# Autodesk Inventor assembly: Ensemble support
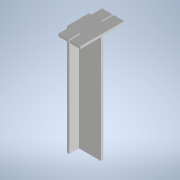
[picture p0: Inventor's stored thumbnail of the model, 180x180]
Saved by Autodesk Inventor 2020 (Build 240168000, 168)
## iProperties
Created: 2019-11-07
Part Number: Ensemble support
Document SubType Name: Assembly
Designer: change_le_nom
Author: change_le_nom
## Documents named in this file (4)
- D:\EIRBOT\Coupe de France 2020\Table de jeu\Support de balise centrale\Ensemble support.iam
- D:\EIRBOT\Coupe de France 2020\Table de jeu\Support de balise centrale\Pièce1.ipt
- D:\EIRBOT\Coupe de France 2020\Table de jeu\Support de balise centrale\Pièce2.ipt
- D:\EIRBOT\Coupe de France 2020\Table de jeu\Support de balise centrale\Pièce3.ipt
## Components (3 placed, 3 different names)
1. Pièce1:1 — Placage:1, Placage:2, Placage:3, Affleurement:1, Affleurement:2, Placage:5, Placage:6
2. Pièce2:1 — Placage:3, Affleurement:1, Affleurement:2, Placage:4
3. Pièce3:1 — Placage:4, Placage:5, Placage:6
## Relationships (8: Mate 6, Flush 2)
- Placage:1 [Mate]: Pièce1:1
- Placage:2 [Mate]: Pièce1:1
- Placage:3 [Mate]: Pièce1:1 ↔ Pièce2:1
- Affleurement:1 [Flush]: Pièce1:1 ↔ Pièce2:1
- Affleurement:2 [Flush] (-89 mm): Pièce1:1 ↔ Pièce2:1
- Placage:4 [Mate]: Pièce2:1 ↔ Pièce3:1
- Placage:5 [Mate]: Pièce1:1 ↔ Pièce3:1
- Placage:6 [Mate] (100 mm): Pièce1:1 ↔ Pièce3:1
